# Autodesk Inventor assembly: L_Unit_SR-I
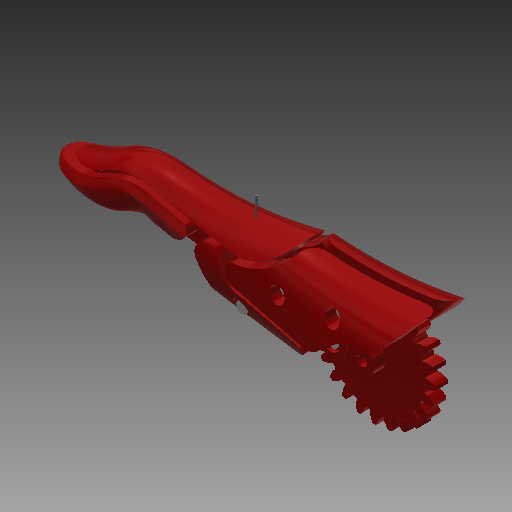
[picture p0: Inventor's stored thumbnail of the model, 512x512]
Saved by Autodesk Inventor 2018.2 (Build 222227000, 227)
## iProperties
Created: 2018-02-15
Part Number: L_Unit_SR-I
Material: 一般
Document SubType Name: Assembly
Designer: sktom
Author: sktom
## Documents named in this file (11)
- D:\CloudStrage\OneDrive\CADMech\HbSizeSMech\UnitHand\Unit_SR-H\Unit_SR-I\L_Unit_SR-I.iam
- D:\CloudStrage\OneDrive\CADMech\HbSizeSMech\UnitHand\Unit_SR-H\Unit_SR-I\L_SR-I-03.ipt
- D:\CloudStrage\OneDrive\CADMech\HbSizeSMech\UnitHand\Unit_SR-H\Unit_SR-I\L_SR-I-02.ipt
- D:\CloudStrage\OneDrive\CADMech\HbSizeSMech\UnitHand\Unit_SR-H\Unit_SR-I\L_SR-I-04.ipt
- D:\CloudStrage\OneDrive\CADMech\HbSizeSMech\UnitHand\Unit_SR-H\Unit_SR-I\L_SR-I-01.ipt
- D:\CloudStrage\OneDrive\CADMech\HbSizeSMech\UnitHand\Unit_SR-H\Unit_SR-I\L_SR-I-05.ipt
- D:\CloudStrage\OneDrive\CADMech\HbSizeSMech\UnitHand\Unit_SR-H\Unit_SR-I\L_SR-I-06.ipt
- D:\CloudStrage\OneDrive\CADMech\HbSizeSMech\UnitHand\Unit_SR-H\Unit_SR-I\L_SR-I-07.ipt
- D:\CloudStrage\OneDrive\CADMech\HbSizeSMech\UnitHand\Unit_SR-H\Unit_SR-I\L_Parts_Screw_M1.4_L6.ipt
- D:\CloudStrage\OneDrive\CADMech\HbSizeSMech\UnitHand\Unit_SR-H\Unit_SR-I\L_Parts_Shaft_Phi1.5_L6.ipt
- D:\CloudStrage\OneDrive\CADMech\HbSizeSMech\UnitHand\Unit_SR-H\Unit_SR-I\L_Parts_TOS 0.3-3-270ﾟ-3.ipt
## Components (16 placed, 10 different names)
1. L_SR-I-03:1 — 挿入:3, 円柱状:1, 回転:4
2. L_SR-I-02:1 — 挿入:3, 挿入:2, 挿入:1, 挿入:4, 挿入:10, 挿入:9
3. L_SR-I-04:1 — 挿入:2, 挿入:1
4. L_SR-I-01:1 — 挿入:4, 挿入:7, 回転:1, 回転:2
5. L_SR-I-05:1 — 挿入:8, 回転:3
6. L_SR-I-06:1 — 挿入:8, 挿入:7, 挿入:6, 挿入:5, 挿入:12, 挿入:11, 円柱状:1
7. L_SR-I-07:1 — 挿入:6, 挿入:5
8. L_Parts_Screw_M1.4_L6:1 — 挿入:12
9. L_Parts_Screw_M1.4_L6:2 — 挿入:11
10. L_Parts_Screw_M1.4_L6:3 — 挿入:10
11. L_Parts_Screw_M1.4_L6:4 — 挿入:9
12. L_Parts_Shaft_Phi1.5_L6:1 — 回転:1
13. L_Parts_Shaft_Phi1.5_L6:2 — 回転:2
14. L_Parts_Shaft_Phi1.5_L6:3 — 回転:4
15. L_Parts_Shaft_Phi1.5_L6:4 — 回転:3
16. L_Parts_TOS 0.3-3-270ﾟ-3:1
## Relationships (17: Insert 12, RevoluteJoint 4, CylindricalJoint 1)
- 挿入:3 [Insert] (0.107 mm): L_SR-I-03:1 ↔ L_SR-I-02:1
- 挿入:2 [Insert]: L_SR-I-02:1 ↔ L_SR-I-04:1
- 挿入:1 [Insert]: L_SR-I-02:1 ↔ L_SR-I-04:1
- 挿入:4 [Insert] (0.145 mm): L_SR-I-02:1 ↔ L_SR-I-01:1
- 挿入:8 [Insert] (0.38 mm): L_SR-I-05:1 ↔ L_SR-I-06:1
- 挿入:7 [Insert] (0.026 mm): L_SR-I-01:1 ↔ L_SR-I-06:1
- 挿入:6 [Insert]: L_SR-I-06:1 ↔ L_SR-I-07:1
- 挿入:5 [Insert]: L_SR-I-06:1 ↔ L_SR-I-07:1
- 挿入:12 [Insert]: L_SR-I-06:1 ↔ L_Parts_Screw_M1.4_L6:1
- 挿入:11 [Insert]: L_SR-I-06:1 ↔ L_Parts_Screw_M1.4_L6:2
- 挿入:10 [Insert]: L_SR-I-02:1 ↔ L_Parts_Screw_M1.4_L6:3
- 挿入:9 [Insert]: L_SR-I-02:1 ↔ L_Parts_Screw_M1.4_L6:4
- 円柱状:1 [CylindricalJoint]: L_SR-I-03:1 ↔ L_SR-I-06:1
- 回転:1 [RevoluteJoint] (-0.725 mm): L_SR-I-01:1 ↔ L_Parts_Shaft_Phi1.5_L6:1
- 回転:2 [RevoluteJoint] (-0.725 mm): L_SR-I-01:1 ↔ L_Parts_Shaft_Phi1.5_L6:2
- 回転:4 [RevoluteJoint]: L_SR-I-03:1 ↔ L_Parts_Shaft_Phi1.5_L6:3
- 回転:3 [RevoluteJoint]: L_SR-I-05:1 ↔ L_Parts_Shaft_Phi1.5_L6:4
